# Autodesk Inventor assembly: MOTOR ARM_exploded
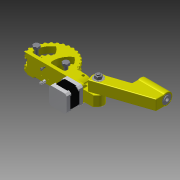
[picture p0: Inventor's stored thumbnail of the model, 180x180]
Saved by Autodesk Inventor 2014 (Build 180170000, 170)
## iProperties
Created: 2013-11-19
Part Number: MOTOR ARM_exploded
Document SubType Name: Assembly
Designer: employee
Author: employee
## Documents named in this file (14)
- C:\Dev\Work\Drukarka\ConceptFORGE\GUS Simpson\INVENTOR FILES\MOTOR ARM_exploded.iam
- C:\Dev\Work\Drukarka\ConceptFORGE\GUS Simpson\INVENTOR FILES\MOTOR ARM.ipt
- C:\Dev\Work\Drukarka\ConceptFORGE\GUS Simpson\INVENTOR FILES\_TUNING PEG.ipt
- C:\Dev\Work\Drukarka\ConceptFORGE\GUS Simpson\INVENTOR FILES\M3x16.ipt
- C:\Dev\Work\Drukarka\ConceptFORGE\GUS Simpson\INVENTOR FILES\M2x10.ipt
- C:\Dev\Work\Drukarka\ConceptFORGE\GUS Simpson\INVENTOR FILES\_SWITCH.ipt
- C:\Dev\Work\Drukarka\ConceptFORGE\GUS Simpson\INVENTOR FILES\M8 NUT.ipt
- C:\Dev\Work\Drukarka\ConceptFORGE\GUS Simpson\INVENTOR FILES\M8x60.ipt
- C:\Dev\Work\Drukarka\ConceptFORGE\GUS Simpson\INVENTOR FILES\M8x55.ipt
- C:\Dev\Work\Drukarka\ConceptFORGE\GUS Simpson\INVENTOR FILES\M8 WASHER.ipt
- C:\Dev\Work\Drukarka\ConceptFORGE\GUS Simpson\INVENTOR FILES\_STEPPER.ipt
- C:\Dev\Work\Drukarka\ConceptFORGE\GUS Simpson\INVENTOR FILES\M3x6.ipt
- C:\Dev\Work\Drukarka\ConceptFORGE\GUS Simpson\INVENTOR FILES\PULLEY.ipt
- C:\Dev\Work\Drukarka\ConceptFORGE\GUS Simpson\INVENTOR FILES\SHOULDER.iam
## Components (23 placed, 13 different names)
1. MOTOR ARM:1 — Insert:1, Angle:1, Insert:2, Insert:4, Insert:5, Insert:8, Insert:9, Insert:10, Insert:11, Angle:2, Angle:3, Angle:4, Angle:5, Insert:14, Angle:6, Insert:15, Angle:7, Insert:17, Angle:8, Insert:18, Insert:19, Insert:20, Insert:21
2. _TUNING PEG:1 — Insert:1, Angle:1, Insert:3
3. M3x16:1 — Insert:2
4. M2x10:1 — Insert:3
5. _SWITCH:1 — Insert:4, Insert:5, Insert:6, Insert:7
6. M2x10:2 — Insert:6
7. M2x10:3 — Insert:7
8. M8 NUT:1 — Insert:8, Angle:4
9. M8 NUT:2 — Insert:10, Angle:3, Insert:12
10. M8 NUT:3 — Insert:9, Angle:5
11. M8 NUT:4 — Insert:11, Angle:2, Insert:13
12. Hex Bolt - Metric M8 x 1.25 x 60:1 — Insert:12
13. Hex Bolt - Metric M8 x 1.25 x 60:2 — Insert:13
14. M8x55:1 — Insert:14, Angle:6
15. M8 WASHER:1 — Insert:15, Insert:16, Insert:23
16. M8 NUT:5 — Insert:16, Angle:7
17. _STEPPER:1 — Insert:17, Angle:8, Insert:22
18. M3x6:1 — Insert:18
19. M3x6:2 — Insert:19
20. M3x6:3 — Insert:20
21. M3x6:4 — Insert:21
22. PULLEY:1 — Insert:22
23. SHOULDER:1 [sub-assembly] — Insert:23
## Relationships (31: Insert 23, Angle 8)
- Insert:1: MOTOR ARM:1 ↔ _TUNING PEG:1
- Angle:1 (0 deg): MOTOR ARM:1 ↔ _TUNING PEG:1
- Insert:2 (6.35 mm): MOTOR ARM:1 ↔ M3x16:1
- Insert:3: _TUNING PEG:1 ↔ M2x10:1
- Insert:4: MOTOR ARM:1 ↔ _SWITCH:1
- Insert:5: MOTOR ARM:1 ↔ _SWITCH:1
- Insert:6: _SWITCH:1 ↔ M2x10:2
- Insert:7: _SWITCH:1 ↔ M2x10:3
- Insert:8: MOTOR ARM:1 ↔ M8 NUT:1
- Insert:9: MOTOR ARM:1 ↔ M8 NUT:3
- Insert:10: MOTOR ARM:1 ↔ M8 NUT:2
- Insert:11: MOTOR ARM:1 ↔ M8 NUT:4
- Angle:2 (0 deg): MOTOR ARM:1 ↔ M8 NUT:4
- Angle:3 (0 deg): MOTOR ARM:1 ↔ M8 NUT:2
- Angle:4 (0 deg): MOTOR ARM:1 ↔ M8 NUT:1
- Angle:5 (0 deg): MOTOR ARM:1 ↔ M8 NUT:3
- Insert:12 (-2 mm): M8 NUT:2 ↔ Hex Bolt - Metric M8 x 1.25 x 60:1
- Insert:13 (-2 mm): M8 NUT:4 ↔ Hex Bolt - Metric M8 x 1.25 x 60:2
- Insert:14: MOTOR ARM:1 ↔ M8x55:1
- Angle:6 (0 deg): MOTOR ARM:1 ↔ M8x55:1
- Insert:15: MOTOR ARM:1 ↔ M8 WASHER:1
- Insert:16 (25 mm): M8 WASHER:1 ↔ M8 NUT:5
- Angle:7 (0 deg): MOTOR ARM:1 ↔ M8 NUT:5
- Insert:17: MOTOR ARM:1 ↔ _STEPPER:1
- Angle:8 (0 deg): MOTOR ARM:1 ↔ _STEPPER:1
- Insert:18: MOTOR ARM:1 ↔ M3x6:1
- Insert:19: MOTOR ARM:1 ↔ M3x6:2
- Insert:20: MOTOR ARM:1 ↔ M3x6:3
- Insert:21: MOTOR ARM:1 ↔ M3x6:4
- Insert:22: _STEPPER:1 ↔ PULLEY:1
- Insert:23: M8 WASHER:1 ↔ SHOULDER:1
